# Autodesk Inventor assembly: plyta_dmd
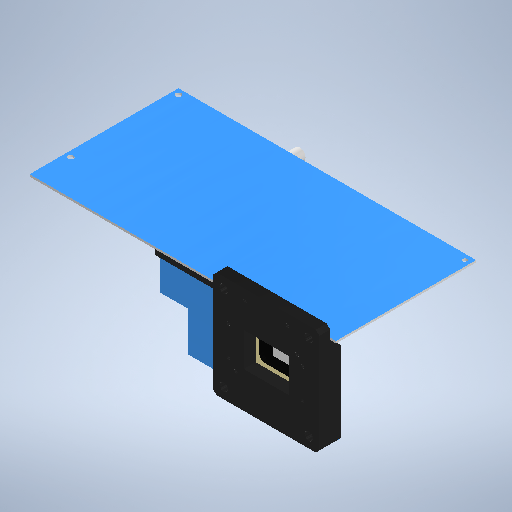
[picture p0: Inventor's stored thumbnail of the model, 512x512]
Saved by Autodesk Inventor 2025.1 (Build 291241020, 241B)
## iProperties
Created: 2024-10-24
Part Number: plyta_dmd
Document SubType Name: Assembly
Designer: PC
Author: PC
## Documents named in this file (8)
- C:\Users\zychlix\Fotolitografia\nowe\plyta_dmd.iam
- electronics_assembly.iam
- C:\Users\zychlix\Fotolitografia\nowe\daughterboard.ipt
- C:\Users\zychlix\Fotolitografia\nowe\motherboard.ipt
- C:\Users\zychlix\Fotolitografia\nowe\podstawka.ipt
- C:\Users\zychlix\Fotolitografia\nowe\DLP.ipt
- C:\Users\zychlix\Fotolitografia\nowe\mocowanie_2000.ipt
- dmd_main_clamp.ipt
## Components (5 placed, 5 different names)
1. daughterboard:1 — Zestawiające:1, Równoległe:1, Zestawiające:2, Zestawiające:3, Zestawiające:4, Zestawiające:5, Równoległe:3, Równoległe:4
2. motherboard:1 — Zestawiające:1, Równoległe:1, Zestawiające:2
3. podstawka:1 — Zestawiające:3, Zestawiające:4, Zestawiające:5, Zestawiające:6, Zestawiające:7, Zestawiające:8
4. DLP:1 — Zestawiające:6, Zestawiające:7, Zestawiające:8
5. dmd_main_clamp:1 — Równoległe:3, Równoległe:4
## Relationships (11: Mate 8, Flush 3)
- Zestawiające:1 [Mate] (1.6 mm): daughterboard:1 ↔ motherboard:1
- Równoległe:1 [Flush] (7 mm): daughterboard:1 ↔ motherboard:1
- Zestawiające:2 [Mate]: daughterboard:1 ↔ motherboard:1
- Zestawiające:3 [Mate]: daughterboard:1 ↔ podstawka:1
- Zestawiające:4 [Mate]: daughterboard:1 ↔ podstawka:1
- Zestawiające:5 [Mate]: daughterboard:1 ↔ podstawka:1
- Zestawiające:6 [Mate]: podstawka:1 ↔ DLP:1
- Zestawiające:7 [Mate]: podstawka:1 ↔ DLP:1
- Zestawiające:8 [Mate]: podstawka:1 ↔ DLP:1
- Równoległe:3 [Flush]: daughterboard:1 ↔ dmd_main_clamp:1
- Równoległe:4 [Flush]: daughterboard:1 ↔ dmd_main_clamp:1
